# Autodesk Inventor assembly: SVWB
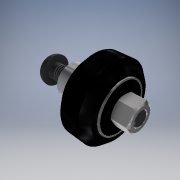
[picture p0: Inventor's stored thumbnail of the model, 180x180]
Saved by Autodesk Inventor 2016 (Build 200138000, 138)
## iProperties
Created: 2016-10-20
Part Number: SVWB
Material: Типовые
Document SubType Name: Assembly
Designer: skhalipa
Author: skhalipa
## Documents named in this file (7)
- C:\Users\skhalipa\Documents\Inventor\SLX-250\SVWB\SVWB.iam
- C:\Users\skhalipa\Documents\Inventor\SLX-250\SVWB\Aluminium spacer 6mm.ipt
- C:\Users\skhalipa\Documents\Inventor\SLX-250\SVWB\Precision Shim 10x5x1.ipt
- C:\Users\skhalipa\Documents\Inventor\SLX-250\SVWB\Solid V Wheel.ipt
- C:\Users\skhalipa\Documents\Inventor\SLX-250\SVWB\ANSI B18.3.4M-M5x0.8x30.ipt
- C:\Users\skhalipa\Documents\Inventor\SLX-250\SVWB\625RS.ipt
- C:\Users\skhalipa\Documents\Inventor\SLX-250\SVWB\Screw M5 GOST 15526-70.ipt
## Components (8 placed, 6 different names)
1. Aluminium spacer 6mm:1 — Вставка:7
2. Precision Shim 10x5x1:1 — Вставка:6, Вставка:7
3. Solid V Wheel:1 — Вставка:2, Вставка:4
4. Винты с полукруглой головкой и шестигранным углублением под ключ - метрическая M5 x 0.8 x 30:1 — Вставка:1
5. 625RS:1 — Вставка:4, Вставка:6
6. 625RS:2 — Вставка:2, Вставка:3, Вставка:5
7. Precision Shim 10x5x1:2 — Вставка:3
8. Гайка ГОСТ 15526-70 M5:1 — Вставка:1, Вставка:5
## Relationships (7: Insert 7)
- Вставка:1 [Insert]: Винты с полукруглой головкой и шестигранным углублением под ключ - метрическая M5 x 0.8 x 30:1 ↔ Гайка ГОСТ 15526-70 M5:1
- Вставка:2 [Insert]: Solid V Wheel:1 ↔ 625RS:2
- Вставка:3 [Insert]: 625RS:2 ↔ Precision Shim 10x5x1:2
- Вставка:4 [Insert]: Solid V Wheel:1 ↔ 625RS:1
- Вставка:5 [Insert]: 625RS:2 ↔ Гайка ГОСТ 15526-70 M5:1
- Вставка:6 [Insert]: Precision Shim 10x5x1:1 ↔ 625RS:1
- Вставка:7 [Insert]: Aluminium spacer 6mm:1 ↔ Precision Shim 10x5x1:1
